# Autodesk Inventor assembly: ASY PRS 9690 Filter legs D1200
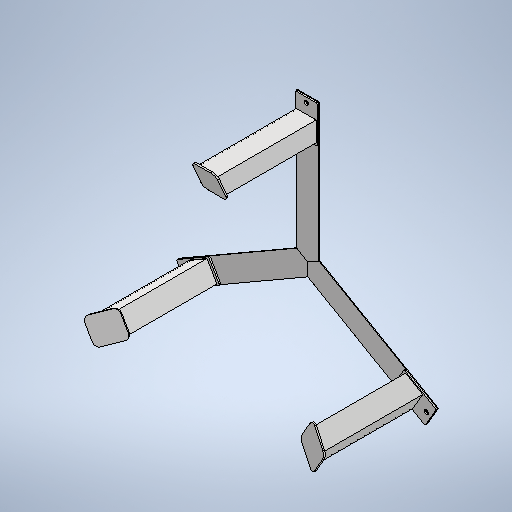
[picture p0: Inventor's stored thumbnail of the model, 512x512]
Saved by Autodesk Inventor 2026.2 (Build 302298010, 298A)
## iProperties
Created: 2025-02-20
Part Number: ASY PRS 9690 Filter legs D1200
Document SubType Name: Assembly
Designer: admin
Mass: 20950.1 g
Surface Area: 14148.6 cm^2
Volume: 2651.55 cm^3
Density: 7.9011 g/cm^3
Author: user
## Documents named in this file (10)
- C:\Users\admin\Documents\Inventor\PRS-Purovsk\ASY PRS 9690 Filter legs D1200.iam
- C:\Users\admin\Documents\Inventor\PRS-Purovsk\PRS 9693 leg sketch_D1200.ipt
- C:\Users\admin\Documents\Inventor\PRS-Purovsk\PRS 9694 leg plate for filter_D1200.ipt
- C:\Users\admin\Documents\Inventor\PRS-Purovsk\PRS 9695 leg floor plate_D1200.ipt
- C:\Users\admin\Documents\Inventor\PRS-Purovsk\PRS 9785 leg floor channel_D1200.ipt
- C:\Users\admin\Documents\Inventor\PRS-Purovsk\PRS 9681 leg tube_D1200.ipt
- C:\Users\admin\Documents\Inventor\PRS-Purovsk\cc\en-US\ISO 7089\ISO 7089 - 16 - 140 HV(1).ipt
- C:\Users\admin\Documents\Inventor\PRS-Purovsk\cc\en-US\ISO 4032(2)\ISO 4032 - M16 - ISO.ipt
- C:\Users\admin\Documents\Inventor\PRS-Purovsk\cc\en-US\ISO 4018\ISO 4018 - M16 x 40.ipt
- C:\Users\admin\Documents\Inventor\PRS-Purovsk\Rps 1696 leg floor pattern.ipt
## Components (23 placed, 9 different names)
1. PRS 9693 leg sketch_D1200:1 — Mate:12
2. PRS 9785 leg floor channel_D1200:1 — Mate:2, Mate:1, Rigid:10
3. ISO 4018 M16 x 40:1
4. ISO 7089 16:1 — Insert:1
5. ISO 4032 M16:1 — Insert:1
6. ISO 4018 M16 x 40:2
7. ISO 4018 M16 x 40:3 — Mate:18
8. ISO 7089 16:2 — Insert:2
9. ISO 7089 16:3 — Mate:24, Insert:3
10. ISO 4032 M16:2 — Insert:2
11. ISO 4032 M16:3 — Insert:3
12. Rps 1696 leg floor pattern:1 — Rigid:2
13. PRS 9681 leg tube_D1200:1 — Mate:7, Flush:1, Mate:8, Mate:9, Mate:10, Mate:12, Mate:13
14. PRS 9695 leg floor plate_D1200:1 — Rigid:10, Mate:7, Flush:1, Mate:8, Mate:18, Mate:24, Rigid:2
15. PRS 9694 leg plate for filter_D1200:1 — Mate:9, Mate:10, Mate:13
16. Rps 1696 leg floor pattern:2
17. PRS 9681 leg tube_D1200:2
18. PRS 9695 leg floor plate_D1200:2
19. PRS 9694 leg plate for filter_D1200:2
20. Rps 1696 leg floor pattern:3
21. PRS 9681 leg tube_D1200:3
22. PRS 9695 leg floor plate_D1200:3
23. PRS 9694 leg plate for filter_D1200:3
## Component patterns: (3 elements, first: Rps 1696 leg floor pattern:1 + PRS 9681 leg tube_D1200:1 + PRS 9695 leg floor plate_D1200:1 + PRS 9694 leg plate for filter_D1200:1)
## Relationships (16: Mate 10, Insert 3, WeldJoint 2, Flush 1)
- Mate:2: PRS 9785 leg floor channel_D1200:1
- Mate:1: PRS 9785 leg floor channel_D1200:1
- Rigid:10 [WeldJoint] (40 mm): PRS 9785 leg floor channel_D1200:1 ↔ PRS 9695 leg floor plate_D1200:1
- Mate:7: PRS 9681 leg tube_D1200:1 ↔ PRS 9695 leg floor plate_D1200:1
- Flush:1 (-10 mm): PRS 9681 leg tube_D1200:1 ↔ PRS 9695 leg floor plate_D1200:1
- Mate:8: PRS 9681 leg tube_D1200:1 ↔ PRS 9695 leg floor plate_D1200:1
- Mate:9: PRS 9681 leg tube_D1200:1 ↔ PRS 9694 leg plate for filter_D1200:1
- Mate:10: PRS 9681 leg tube_D1200:1 ↔ PRS 9694 leg plate for filter_D1200:1
- Mate:12: PRS 9693 leg sketch_D1200:1 ↔ PRS 9681 leg tube_D1200:1
- Mate:13: PRS 9681 leg tube_D1200:1 ↔ PRS 9694 leg plate for filter_D1200:1
- Mate:18: ISO 4018 M16 x 40:3 ↔ PRS 9695 leg floor plate_D1200:1
- Mate:24: ISO 7089 16:3 ↔ PRS 9695 leg floor plate_D1200:1
- Insert:1: ISO 7089 16:1 ↔ ISO 4032 M16:1
- Insert:2: ISO 7089 16:2 ↔ ISO 4032 M16:2
- Insert:3: ISO 7089 16:3 ↔ ISO 4032 M16:3
- Rigid:2 [WeldJoint]: Rps 1696 leg floor pattern:1 ↔ PRS 9695 leg floor plate_D1200:1
## Named parameters: Out_diam = 963 mm
